# Autodesk Inventor assembly: Carro 8.5
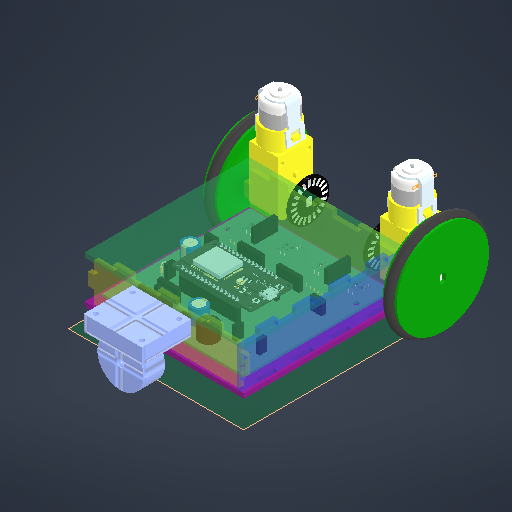
[picture p0: Inventor's stored thumbnail of the model, 512x512]
Saved by Autodesk Inventor 2026 (Build 300175000, 175)
## iProperties
Created: 2025-11-06
Part Number: Carro 8.5
Document SubType Name: Assembly
Designer: pregu
Author: pregu
## Documents named in this file (11)
- C:\Users\pregu\OneDrive\Documentos\Carro 8.5\Carro 8.5.iam
- C:\Users\pregu\OneDrive\Documentos\Carro 8.5\Esp_pcb.iam
- C:\Users\pregu\OneDrive\Documentos\Carro 8.5\Chassi_inf.ipt
- C:\Users\pregu\OneDrive\Documentos\Carro 8.5\Acrilico-Parachoque-Parede-Inf.ipt
- C:\Users\pregu\OneDrive\Documentos\Carro 8.5\Acrilico-Parachoque.ipt
- C:\Users\pregu\OneDrive\Documentos\Carro 8.5\Chassi_mid.ipt
- C:\Users\pregu\OneDrive\Documentos\Carro 8.5\Motor Amarelo\Motor.iam
- C:\Users\pregu\OneDrive\Documentos\Carro 8.5\MTG eixorodaencode.iam
- C:\Users\pregu\OneDrive\Documentos\Carro 8.5\Motor Amarelo\Motor_MIR.iam
- C:\Users\pregu\OneDrive\Documentos\Carro 8.5\Roda-boba.0001.ipt
- C:\Users\pregu\OneDrive\Documentos\Carro 8.5\MTG eixorodaencode_MIR1.iam
## Components (12 placed, 10 different names)
1. Esp_pcb:1 [sub-assembly] — Coincidente:1, Coincidente:5, Coincidente:6, Alinhado:1, Coincidente:8, Coincidente:11, Coincidente:13
2. Chassi_inf:1 — Coincidente:1, Coincidente:6, Alinhado:1, Alinhado:2, Coincidente:7, Coincidente:10, Alinhado:3, Coincidente:12, Coincidente:14, Alinhado:4, Simetria:1, Coincidente:17, Coincidente:18, Alinhado:9
3. Acrilico-Parachoque-Parede-Inf:1 — Coincidente:5, Alinhado:2, Coincidente:7, Coincidente:9, Coincidente:15, Alinhado:5
4. Acrilico-Parachoque:1 — Coincidente:8, Coincidente:9, Coincidente:10, Coincidente:16
5. Acrilico-Parachoque-Parede-Inf:2 — Coincidente:11, Alinhado:3, Coincidente:12
6. Acrilico-Parachoque:2 — Coincidente:13, Coincidente:14, Coincidente:15
7. Chassi_mid:1 — Coincidente:16, Alinhado:4, Alinhado:5, Simetria:1, Alinhado:8, Coincidente:19, Coincidente:20, Alinhado:10
8. Roda-boba.0001:1 — Coincidente:19, Coincidente:20, Alinhado:10
9. Motor:1 [sub-assembly] — Inserir:1, Coincidente:17, Coincidente:18, Alinhado:9
10. MTG eixorodaencode:1 [sub-assembly] — Inserir:1
11. Motor_MIR:1 [sub-assembly]
12. MTG eixorodaencode_MIR1:1 [sub-assembly]
## Component patterns: (2 elements, first: Motor:1 + MTG eixorodaencode:1)
## Relationships (27: Mate 17, Flush 8, Insert 1, Symmetry 1)
- Coincidente:1 [Mate] (3 mm): Esp_pcb:1 ↔ Chassi_inf:1
- Coincidente:5 [Mate] (1.25 mm): Esp_pcb:1 ↔ Acrilico-Parachoque-Parede-Inf:1
- Coincidente:6 [Mate] (-5.75 mm): Esp_pcb:1 ↔ Chassi_inf:1
- Alinhado:1 [Flush] (-5.75 mm): Esp_pcb:1 ↔ Chassi_inf:1
- Alinhado:2 [Flush]: Chassi_inf:1 ↔ Acrilico-Parachoque-Parede-Inf:1
- Coincidente:7 [Mate]: Chassi_inf:1 ↔ Acrilico-Parachoque-Parede-Inf:1
- Coincidente:8 [Mate] (1.25 mm): Esp_pcb:1 ↔ Acrilico-Parachoque:1
- Coincidente:9 [Mate]: Acrilico-Parachoque-Parede-Inf:1 ↔ Acrilico-Parachoque:1
- Coincidente:10 [Mate]: Chassi_inf:1 ↔ Acrilico-Parachoque:1
- Coincidente:11 [Mate] (1.25 mm): Esp_pcb:1 ↔ Acrilico-Parachoque-Parede-Inf:2
- Alinhado:3 [Flush]: Chassi_inf:1 ↔ Acrilico-Parachoque-Parede-Inf:2
- Coincidente:12 [Mate]: Chassi_inf:1 ↔ Acrilico-Parachoque-Parede-Inf:2
- Coincidente:13 [Mate] (1.25 mm): Esp_pcb:1 ↔ Acrilico-Parachoque:2
- Coincidente:14 [Mate]: Chassi_inf:1 ↔ Acrilico-Parachoque:2
- Coincidente:15 [Mate]: Acrilico-Parachoque-Parede-Inf:1 ↔ Acrilico-Parachoque:2
- Coincidente:16 [Mate]: Acrilico-Parachoque:1 ↔ Chassi_mid:1
- Alinhado:4 [Flush]: Chassi_inf:1 ↔ Chassi_mid:1
- Alinhado:5 [Flush]: Acrilico-Parachoque-Parede-Inf:1 ↔ Chassi_mid:1
- Inserir:1: Motor:1 ↔ MTG eixorodaencode:1
- Simetria:1 [Symmetry]: Chassi_inf:1 ↔ Chassi_mid:1
- Alinhado:8 [Flush] (40 mm): Chassi_mid:1
- Coincidente:17 [Mate]: Chassi_inf:1 ↔ Motor:1
- Coincidente:18 [Mate]: Chassi_inf:1 ↔ Motor:1
- Alinhado:9 [Flush]: Chassi_inf:1 ↔ Motor:1
- Coincidente:19 [Mate]: Chassi_mid:1 ↔ Roda-boba.0001:1
- Coincidente:20 [Mate]: Chassi_mid:1 ↔ Roda-boba.0001:1
- Alinhado:10 [Flush] (31.25 mm): Chassi_mid:1 ↔ Roda-boba.0001:1
